# Autodesk Inventor assembly: цепь
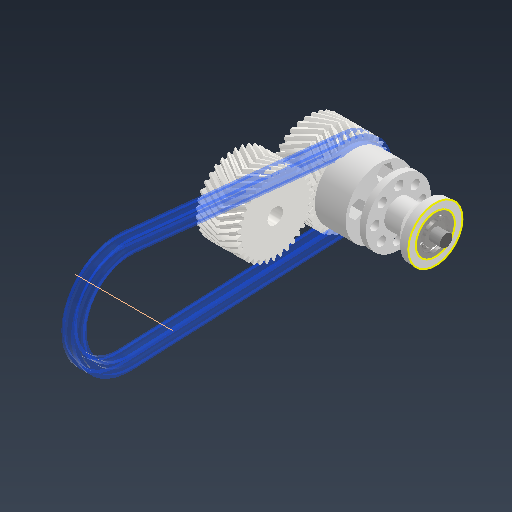
[picture p0: Inventor's stored thumbnail of the model, 512x512]
Saved by Autodesk Inventor 2025.2 (Build 292293000, 293)
## iProperties
Created: 2024-07-09
Part Number: цепь
Document SubType Name: Assembly
Designer: Phantom
Author: Phantom
## Documents named in this file (7)
- F:\Phantom16950\цепь.iam
- F:\Phantom16950\Цепной привод2.iam
- F:\Phantom16950\втулка для подш 2 часть.ipt
- F:\Phantom16950\втулка для подш.ipt
- F:\Phantom16950\Деталь_64.ipt
- F:\Phantom16950\BS 290 SKF - SKF 626-RZ.ipt
- F:\Phantom16950\цепь\Мастер проектирования\Цилиндрическое зубчатое зацепление4.iam
## Components (7 placed, 6 different names)
1. Цепной привод:1 [sub-assembly] — Совмещение:22, Совмещение:24, Заподлицо:4
2. втулка для подш 2 часть:1 — Совмещение:16, Совмещение:20, Совмещение:23
3. втулка для подш:1 — Совмещение:16, Совмещение:17, Совмещение:22, Совмещение:24, Заподлицо:4, Совмещение:25, Совмещение:26
4. Деталь_64:1 — Совмещение:17, Совмещение:19, Совмещение:21, Совмещение:23
5. BS 290 SKF - SKF 626-RZ:1 — Совмещение:20, Совмещение:21
6. BS 290 SKF - SKF 626-RZ:2 — Совмещение:19, Совмещение:27
7. Цилиндрическое зубчатое зацепление:4 [sub-assembly] — Совмещение:25, Совмещение:26, Совмещение:27
## Relationships (12: Mate 11, Flush 1)
- Совмещение:16 [Mate]: втулка для подш 2 часть:1 ↔ втулка для подш:1
- Совмещение:17 [Mate]: втулка для подш:1 ↔ Деталь_64:1
- Совмещение:19 [Mate]: Деталь_64:1 ↔ BS 290 SKF - SKF 626-RZ:2
- Совмещение:20 [Mate]: втулка для подш 2 часть:1 ↔ BS 290 SKF - SKF 626-RZ:1
- Совмещение:21 [Mate]: Деталь_64:1 ↔ BS 290 SKF - SKF 626-RZ:1
- Совмещение:22 [Mate]: Цепной привод:1 ↔ втулка для подш:1
- Совмещение:23 [Mate]: втулка для подш 2 часть:1 ↔ Деталь_64:1
- Совмещение:24 [Mate]: Цепной привод:1 ↔ втулка для подш:1
- Заподлицо:4 [Flush] (4 mm): Цепной привод:1 ↔ втулка для подш:1
- Совмещение:25 [Mate]: втулка для подш:1 ↔ Цилиндрическое зубчатое зацепление:4
- Совмещение:26 [Mate]: втулка для подш:1 ↔ Цилиндрическое зубчатое зацепление:4
- Совмещение:27 [Mate]: BS 290 SKF - SKF 626-RZ:2 ↔ Цилиндрическое зубчатое зацепление:4
